# Autodesk Inventor assembly: finalStagesAssembly
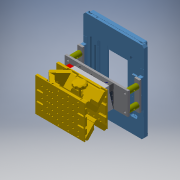
[picture p0: Inventor's stored thumbnail of the model, 180x180]
Saved by Autodesk Inventor 2016 (Build 200138000, 138)
## iProperties
Created: 2016-10-04
Part Number: finalStagesAssembly
Document SubType Name: Assembly
Designer: sims01
Author: sims01
## Documents named in this file (9)
- H:\Documents\LSFM_3\setup\mechanical\design\stagesAssemblyFinal\finalStagesAssembly.iam
- H:\Documents\LSFM_3\setup\mechanical\design\stagesAssemblyFinal\newportHighLoadJack.ipt
- H:\Documents\LSFM_3\setup\mechanical\design\stagesAssemblyFinal\zStageJackAttach_piece1.ipt
- H:\Documents\LSFM_3\setup\mechanical\design\stagesAssemblyFinal\zStageJackAttach_piece2.ipt
- H:\Documents\LSFM_3\setup\mechanical\design\stagesAssemblyFinal\piStage_Z.ipt
- H:\Documents\LSFM_3\setup\mechanical\design\stagesAssemblyFinal\zStagePostAttach.ipt
- H:\Documents\LSFM_3\setup\mechanical\design\stagesAssemblyFinal\xyStagePostAttach.ipt
- H:\Documents\LSFM_3\setup\mechanical\design\stagesAssemblyFinal\piStage_XY.ipt
- H:\Documents\LSFM_3\setup\mechanical\design\stagesAssemblyFinal\50mmPost.ipt
## Components (12 placed, 8 different names)
1. newportHighLoadJack:1 — Rigid:1, Rigid:2
2. zStageJackAttach_piece1:1 — Rigid:2, Rigid:3
3. zStageJackAttach_piece2:2 — Rigid:1
4. piStage_Z:2 — Rigid:3, Rigid:4
5. zStagePostAttach:1 — Rigid:4, Rigid:12, Rigid:13, Rigid:14, Rigid:15
6. xyStagePostAttach:1 — Rigid:11, Mate:2
7. xyStagePostAttach:2 — Mate:1
8. piStage_XY:1 — Rigid:11
9. 50mmPost:1 — Rigid:12
10. 50mmPost:2 — Rigid:13, Mate:1
11. 50mmPost:3 — Rigid:15
12. 50mmPost:4 — Rigid:14, Mate:2
## Relationships (11: WeldJoint 9, Mate 2)
- Rigid:1 [WeldJoint]: newportHighLoadJack:1 ↔ zStageJackAttach_piece2:2
- Rigid:2 [WeldJoint]: newportHighLoadJack:1 ↔ zStageJackAttach_piece1:1
- Rigid:3 [WeldJoint]: zStageJackAttach_piece1:1 ↔ piStage_Z:2
- Rigid:4 [WeldJoint]: piStage_Z:2 ↔ zStagePostAttach:1
- Rigid:11 [WeldJoint]: xyStagePostAttach:1 ↔ piStage_XY:1
- Rigid:12 [WeldJoint]: zStagePostAttach:1 ↔ 50mmPost:1
- Rigid:13 [WeldJoint]: zStagePostAttach:1 ↔ 50mmPost:2
- Rigid:14 [WeldJoint]: zStagePostAttach:1 ↔ 50mmPost:4
- Rigid:15 [WeldJoint]: zStagePostAttach:1 ↔ 50mmPost:3
- Mate:1: xyStagePostAttach:2 ↔ 50mmPost:2
- Mate:2: xyStagePostAttach:1 ↔ 50mmPost:4
